# Autodesk Inventor assembly: Hand
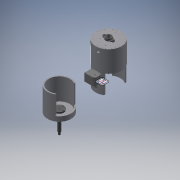
[picture p0: Inventor's stored thumbnail of the model, 180x180]
Saved by Autodesk Inventor 2016 (Build 200138000, 138)
## iProperties
Created: 2016-11-12
Part Number: Hand
Material: 一般
Document SubType Name: Assembly
Designer: Daisuke
Author: Daisuke
## Documents named in this file (4)
- C:\Users\Daisuke\Documents\GitHub\CAD\Hand\ver1\Hand.iam
- C:\Users\Daisuke\Documents\GitHub\CAD\Hand\ver1\insideHand.iam
- C:\Users\Daisuke\Documents\GitHub\CAD\Hand\ver1\outsideHand.iam
- C:\Users\Daisuke\Documents\GitHub\CAD\Hand\ver1\Servo.iam
## Components (3 placed, 3 different names)
1. insideHand:1 [sub-assembly]
2. outsideHand:1 [sub-assembly] — 挿入:1, 挿入:2
3. Servo:1 [sub-assembly] — 挿入:1, 挿入:2
## Relationships (2: Insert 2)
- 挿入:1 [Insert]: outsideHand:1 ↔ Servo:1
- 挿入:2 [Insert]: outsideHand:1 ↔ Servo:1
